# Autodesk Inventor assembly: pairofwheels
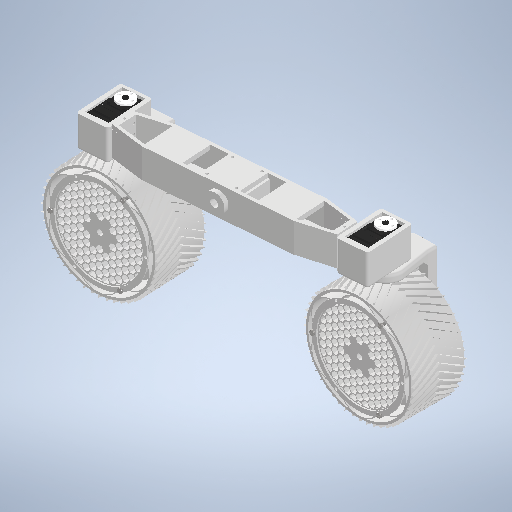
[picture p0: Inventor's stored thumbnail of the model, 512x512]
Saved by Autodesk Inventor 2025.3 (Build 293356000, 356)
## iProperties
Created: 2026-04-12
Part Number: pairofwheels
Document SubType Name: Assembly
Designer: ksawe
Author: ksawe
## Documents named in this file (5)
- C:\Users\ksawe\OneDrive\Pulpit\Exomy v1\wersja2\pairofwheels.iam
- C:\Users\ksawe\OneDrive\Pulpit\Exomy v1\wersja2\basketwheel.iam
- C:\Users\ksawe\OneDrive\Pulpit\Exomy v1\wersja2\pret_handler_v2.ipt
- C:\Users\ksawe\OneDrive\Pulpit\Exomy v1\wersja2\wheelbasketleft.iam
- C:\Users\ksawe\OneDrive\Pulpit\Exomy v1\wersja2\nakladka.ipt
## Components (4 placed, 4 different names)
1. basketwheel:1 [sub-assembly] — Mate:1, Mate:2, Mate:3
2. pret_handler_v2:1 — Mate:1, Mate:2, Mate:3, Mate:4, Mate:5, Mate:6, Mate:7, Mate:8
3. wheelbasketleft:1 [sub-assembly] — Mate:4, Mate:5
4. nakladka:1 — Mate:6, Mate:7, Mate:8
## Relationships (8: Mate 8)
- Mate:1: basketwheel:1 ↔ pret_handler_v2:1
- Mate:2: basketwheel:1 ↔ pret_handler_v2:1
- Mate:3: basketwheel:1 ↔ pret_handler_v2:1
- Mate:4: pret_handler_v2:1 ↔ wheelbasketleft:1
- Mate:5: pret_handler_v2:1 ↔ wheelbasketleft:1
- Mate:6: pret_handler_v2:1 ↔ nakladka:1
- Mate:7: pret_handler_v2:1 ↔ nakladka:1
- Mate:8: pret_handler_v2:1 ↔ nakladka:1
